# Autodesk Inventor assembly: Chain Testing
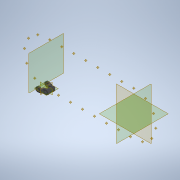
[picture p0: Inventor's stored thumbnail of the model, 180x180]
Saved by Autodesk Inventor 2020 (Build 240168000, 168)
## iProperties
Created: 2019-09-16
Part Number: Chain Testing
Document SubType Name: Assembly
Designer: Corey
Author: Corey
## Documents named in this file (3)
- C:\Users\Corey\Documents\Tower-Takeover-CAD\Chain Testing.iam
- C:\Users\Corey\Documents\Tower-Takeover-CAD\Chain Sketch.ipt
- C:\Users\Corey\Documents\Tower-Takeover-CAD\Parts\Motion\Chain & Tank Tread\Chain Link.ipt
## Components (2 placed, 2 different names)
1. Chain Sketch:1 — Mate:1, Mate:2, Mate:3, Flush:1, Mate:4
2. Chain Link:1 — Mate:3, Flush:1, Mate:4
## Relationships (5: Mate 4, Flush 1)
- Mate:1: Chain Sketch:1
- Mate:2: Chain Sketch:1
- Mate:3: Chain Sketch:1 ↔ Chain Link:1
- Flush:1 (-12.7 mm): Chain Sketch:1 ↔ Chain Link:1
- Mate:4: Chain Sketch:1 ↔ Chain Link:1
